# Autodesk Inventor assembly: Assembly3
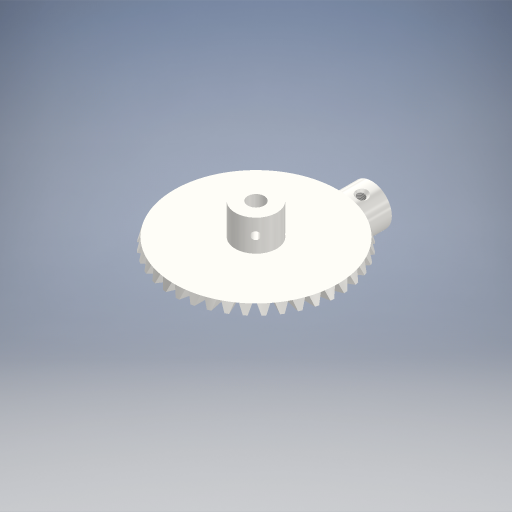
[picture p0: Inventor's stored thumbnail of the model, 512x512]
Saved by Autodesk Inventor 2024 (Build 280153000, 153)
## iProperties
Created: 2024-04-13
Part Number: Assembly3
Document SubType Name: Assembly
Designer: Alex
Author: Alex
## Documents named in this file (2)
- C:\Shared\alex-bartella-schoolwork\4z03\final\Assembly3.iam
- C:\Shared\alex-bartella-schoolwork\4z03\final\final\gears\Bevel Gears4.iam
## Components (1 placed, 1 different names)
1. Bevel Gears:1 [sub-assembly] — Mate:1, Mate:2
## Relationships (2: Mate 2)
- Mate:1: Bevel Gears:1
- Mate:2: Bevel Gears:1
